# Autodesk Inventor assembly: Hose Assembly
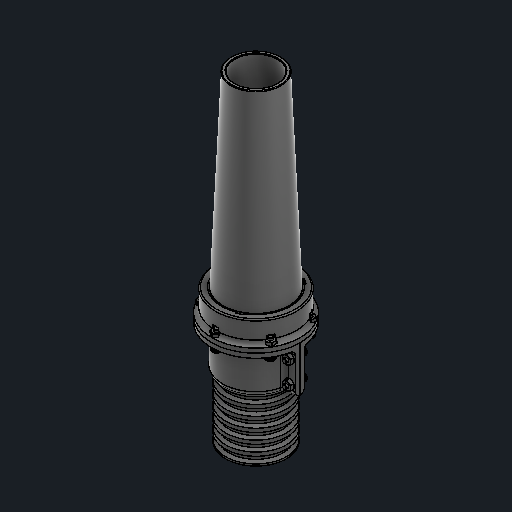
[picture p0: Inventor's stored thumbnail of the model, 512x512]
Saved by Autodesk Inventor 2026.2 (Build 302298000, 298)
## iProperties
Created: 2026-07-12
Part Number: Hose Assembly
Document SubType Name: Assembly
Designer: JoshuaEah
Author: JoshuaEah
## Documents named in this file (7)
- C:\Users\JoshuaEah\Documents\GitHub\Designed-Trinkets\Makera Carvera Air\Air Port\40mm Vacuum Hose Adapter\Assemblies\Nozzle Side Assembly.iam
- C:\Users\JoshuaEah\Documents\GitHub\Designed-Trinkets\Makera Carvera Air\Air Port\40mm Vacuum Hose Adapter\Parts\Flanged Hose Fitting.ipt
- C:\Users\JoshuaEah\Documents\GitHub\Designed-Trinkets\Makera Carvera Air\Air Port\40mm Vacuum Hose Adapter\Parts\40mm Vacuum Hose.ipt
- C:\Users\JoshuaEah\Documents\GitHub\Designed-Trinkets\Makera Carvera Air\Air Port\40mm Vacuum Hose Adapter\Hardware\M3x10 SHCS.ipt
- C:\Users\JoshuaEah\Documents\GitHub\Designed-Trinkets\Makera Carvera Air\Air Port\40mm Vacuum Hose Adapter\Hardware\M3x0.5 Hex Nut.ipt
- C:\Users\JoshuaEah\Documents\GitHub\Designed-Trinkets\Makera Carvera Air\Air Port\40mm Vacuum Hose Adapter\Parts\Vacuum Attachments\Flanged Attachment Mount.ipt
- C:\Users\JoshuaEah\Documents\GitHub\Designed-Trinkets\Makera Carvera Air\Air Port\40mm Vacuum Hose Adapter\Parts\Vacuum Attachments\Basic Vacuum Nozzle.ipt
## Components (25 placed, 6 different names)
1. Flanged Hose Fitting:1 — Insert:1, Insert:2, Insert:3, Insert:6, Insert:7, Insert:10, Insert:11, Insert:16
2. Flanged Hose Fitting:2 — Insert:1, Insert:2, Insert:4, Insert:5, Insert:8, Insert:9, Insert:15, Insert:14
3. 40mm Vacuum Hose:1 — Insert:3
4. M3x10 SHCS:1 — Insert:4
5. M3x10 SHCS:2 — Insert:5
6. M3x10 SHCS:3 — Insert:6
7. M3x10 SHCS:4 — Insert:7
8. M3x0.5 Hex Nut:1 — Insert:8
9. M3x0.5 Hex Nut:2 — Insert:9
10. M3x0.5 Hex Nut:3 — Insert:10
11. M3x0.5 Hex Nut:4 — Insert:11
12. Flanged Attachment Mount:1 — Insert:15, Insert:16, Insert:17, Mate:1, Mate:2
13. Basic Vacuum Nozzle:1 — Mate:1, Mate:2
14. M3x10 SHCS:5 — Insert:14
15. M3x0.5 Hex Nut:5 — Insert:17
16. M3x10 SHCS:6
17. M3x0.5 Hex Nut:6
18. M3x10 SHCS:7
19. M3x0.5 Hex Nut:7
20. M3x10 SHCS:8
21. M3x0.5 Hex Nut:8
22. M3x10 SHCS:9
23. M3x0.5 Hex Nut:9
24. M3x10 SHCS:10
25. M3x0.5 Hex Nut:10
## Component patterns: Flange Mounting Hardware (6 elements)
## Relationships (17: Insert 15, Mate 2)
- Insert:1: Flanged Hose Fitting:1 ↔ Flanged Hose Fitting:2
- Insert:2: Flanged Hose Fitting:1 ↔ Flanged Hose Fitting:2
- Insert:3 (0.1 mm): Flanged Hose Fitting:1 ↔ 40mm Vacuum Hose:1
- Insert:4: Flanged Hose Fitting:2 ↔ M3x10 SHCS:1
- Insert:5: Flanged Hose Fitting:2 ↔ M3x10 SHCS:2
- Insert:6: Flanged Hose Fitting:1 ↔ M3x10 SHCS:3
- Insert:7: Flanged Hose Fitting:1 ↔ M3x10 SHCS:4
- Insert:8: Flanged Hose Fitting:2 ↔ M3x0.5 Hex Nut:1
- Insert:9: Flanged Hose Fitting:2 ↔ M3x0.5 Hex Nut:2
- Insert:10: Flanged Hose Fitting:1 ↔ M3x0.5 Hex Nut:3
- Insert:11: Flanged Hose Fitting:1 ↔ M3x0.5 Hex Nut:4
- Insert:14: Flanged Hose Fitting:2 ↔ M3x10 SHCS:5
- Insert:15: Flanged Hose Fitting:2 ↔ Flanged Attachment Mount:1
- Insert:16: Flanged Hose Fitting:1 ↔ Flanged Attachment Mount:1
- Insert:17: Flanged Attachment Mount:1 ↔ M3x0.5 Hex Nut:5
- Mate:1: Flanged Attachment Mount:1 ↔ Basic Vacuum Nozzle:1
- Mate:2: Flanged Attachment Mount:1 ↔ Basic Vacuum Nozzle:1
